# Autodesk Inventor assembly: Reser Button
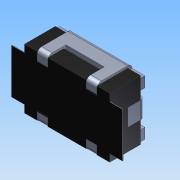
[picture p0: Inventor's stored thumbnail of the model, 180x180]
Saved by Autodesk Inventor 2016 (Build 200138000, 138)
## iProperties
Created: 2017-12-12
Part Number: Reser Button
Document SubType Name: Assembly
Designer: User
Mass: 0.0198932 g
Surface Area: 0.881355 cm^2
Volume: 0.0198932 cm^3
Density: 1 g/cm^3
Author: User
## Documents named in this file (3)
- E:\_Project TANK\Purchased\Arduino\Arduino NANO\Reser Button.iam
- E:\_Project TANK\Purchased\Arduino\Arduino NANO\User Library-arduino_nano\User Library-arduino_nano_reset core.ipt
- E:\_Project TANK\Purchased\Arduino\Arduino NANO\User Library-arduino_nano\User Library-arduino_nano_reset shell.ipt
## Components (2 placed, 2 different names)
1. User Library-arduino_nano_reset core:1 — Flush:1, Flush:2, Flush:3, Insert:1, Mate:1
2. User Library-arduino_nano_reset shell:1 — Insert:1, Mate:1
## Relationships (5: Flush 3, Insert 1, Mate 1)
- Flush:1: User Library-arduino_nano_reset core:1
- Flush:2: User Library-arduino_nano_reset core:1
- Flush:3: User Library-arduino_nano_reset core:1
- Insert:1: User Library-arduino_nano_reset core:1 ↔ User Library-arduino_nano_reset shell:1
- Mate:1: User Library-arduino_nano_reset core:1 ↔ User Library-arduino_nano_reset shell:1
